# Autodesk Inventor assembly: cupula_partes_2
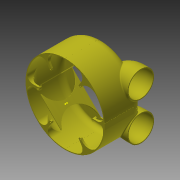
[picture p0: Inventor's stored thumbnail of the model, 180x180]
Saved by Autodesk Inventor 2015 (Build 190159000, 159)
## iProperties
Created: 2015-06-04
Part Number: cupula_partes_2
Document SubType Name: Assembly
Designer: david_000
Author: david_000
## Documents named in this file (5)
- C:\Users\david_000\Desktop\minibot-code\mechanics\cupula_partes_2.iam
- C:\Users\david_000\Desktop\minibot-code\mechanics\cupula2_parte_delantera.ipt
- C:\Users\david_000\Desktop\minibot-code\mechanics\cupula2_parte_delantera_2.ipt
- C:\Users\david_000\Desktop\minibot-code\mechanics\base_trasera_2_espejo.ipt
- C:\Users\david_000\Desktop\minibot-code\mechanics\base_trasera_2.ipt
## Components (4 placed, 4 different names)
1. cupula2_parte_delantera:1 — Coincidencia:1, Coincidencia:2, Nivelación:1, Coincidencia:6, Nivelación:2, Coincidencia:7
2. cupula2_parte_delantera_2:1 — Coincidencia:1, Coincidencia:2, Nivelación:1
3. base_trasera_2_espejo:1 — Coincidencia:3, Coincidencia:4, Coincidencia:5
4. base_trasera_2:1 — Coincidencia:3, Coincidencia:4, Coincidencia:5, Coincidencia:6, Nivelación:2, Coincidencia:7
## Relationships (9: Mate 7, Flush 2)
- Coincidencia:1 [Mate]: cupula2_parte_delantera:1 ↔ cupula2_parte_delantera_2:1
- Coincidencia:2 [Mate]: cupula2_parte_delantera:1 ↔ cupula2_parte_delantera_2:1
- Nivelación:1 [Flush]: cupula2_parte_delantera:1 ↔ cupula2_parte_delantera_2:1
- Coincidencia:3 [Mate]: base_trasera_2_espejo:1 ↔ base_trasera_2:1
- Coincidencia:4 [Mate]: base_trasera_2_espejo:1 ↔ base_trasera_2:1
- Coincidencia:5 [Mate]: base_trasera_2_espejo:1 ↔ base_trasera_2:1
- Coincidencia:6 [Mate]: cupula2_parte_delantera:1 ↔ base_trasera_2:1
- Nivelación:2 [Flush]: cupula2_parte_delantera:1 ↔ base_trasera_2:1
- Coincidencia:7 [Mate]: cupula2_parte_delantera:1 ↔ base_trasera_2:1
